# Autodesk Inventor assembly: astra
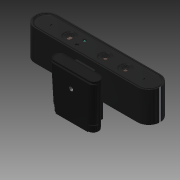
[picture p0: Inventor's stored thumbnail of the model, 180x180]
Saved by Autodesk Inventor 2015 (Build 190159000, 159)
## iProperties
Created: 2016-02-10
Part Number: astra
Document SubType Name: Assembly
Designer: John
Author: John
## Documents named in this file (4)
- C:\Users\John\Desktop\Orbbec Astra S\astra.iam
- C:\Users\John\Desktop\Orbbec Astra S\Astra.ipt
- C:\Users\John\Desktop\Orbbec Astra S\astra_clip1.ipt
- C:\Users\John\Desktop\Orbbec Astra S\astra_clip2.ipt
## Components (3 placed, 3 different names)
1. Astra:1 — Mate:1, Mate:2
2. astra_clip1:1 — Mate:1, Mate:2, Mate:3, Mate:4
3. astra_clip2:1 — Mate:3, Mate:4
## Relationships (4: Mate 4)
- Mate:1: Astra:1 ↔ astra_clip1:1
- Mate:2: Astra:1 ↔ astra_clip1:1
- Mate:3: astra_clip1:1 ↔ astra_clip2:1
- Mate:4: astra_clip1:1 ↔ astra_clip2:1
